# Autodesk Inventor assembly: Carriage
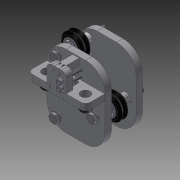
[picture p0: Inventor's stored thumbnail of the model, 180x180]
Saved by Autodesk Inventor 2014 (Build 180170000, 170)
## iProperties
Created: 2014-08-27
Part Number: Carriage
Document SubType Name: Assembly
Designer: ThatOtherGuy
Author: ThatOtherGuy
## Documents named in this file (17)
- U:\Hobbies\Inventor\KosselCNC1515\Carriage\Carriage.iam
- U:\Hobbies\Inventor\KosselCNC1515\Carriage\Carriage_Frame.ipt
- U:\Hobbies\Inventor\KosselCNC1515\Carriage\Carriage_Spacer-6.35mm.ipt
- Carriage_Spacer-6.35mm.ipt
- U:\Hobbies\Inventor\KosselCNC1515\Carriage\OpenVWheel.iam
- U:\Hobbies\Inventor\Content Center Files\R2014\en-US\DIN 125-1  A\DIN 125 - A 5.3.ipt
- U:\Hobbies\Inventor\Content Center Files\R2014\en-US\DIN 125-1  A\DIN 125 - A 4.3.ipt
- U:\Hobbies\Inventor\Content Center Files\R2014\en-US\ISO 10511\ISO 10511 - M5.ipt
- U:\Hobbies\Inventor\KosselCNC1515\Carriage\Carriage_Frame_Back.ipt
- U:\Hobbies\Inventor\KosselCNC1515\Carriage\Carriage_Joint_Frame.ipt
- U:\Hobbies\Inventor\KosselCNC1515\Joints\Joint_Ball_Bearing_12MM.ipt
- U:\Hobbies\Inventor\Content Center Files\R2014\en-US\JIS B 1180  A\JIS B 1180 - A M5 x 50 - 0.8.ipt
- U:\Hobbies\Inventor\KosselCNC1515\Carriage\Carriage_Joint_Boltblock.ipt
- U:\Hobbies\Inventor\KosselCNC1515\Carriage\Carriage_Joint_Boltblock_Brace.ipt
- U:\Hobbies\Inventor\Content Center Files\R2014\en-US\ANSI B18.3.1M(1)\ANSI B18.3.1M - M3x0.5 x 25(2).ipt
- U:\Hobbies\Inventor\Content Center Files\R2014\en-US\DIN 934\DIN 934 - M3 x 0.5.ipt
- U:\Hobbies\Inventor\KosselCNC1515\Carriage\OpenBuilds_Eccentric_Spacer.ipt
## Components (38 placed, 15 different names)
1. Carriage_Frame_Back:1 — Mate:1, Mate:2, Mate:3, Mate:4, Insert:6, Insert:7, Mate:50, Mate:65
2. Carriage_Frame:2 — Mate:26, Mate:27, Mate:28, Insert:4, Insert:5, Mate:45, Mate:46, Mate:60, Mate:65
3. Carriage_Joint_Frame:1 — Mate:45, Mate:46, Mate:60, Mate:71, Mate:72, Tangent:1, Tangent:2, Mate:75, Mate:76, Mate:77
4. Joint_Ball_Bearing_12MM:1 — Mate:71, Tangent:1
5. Joint_Ball_Bearing_12MM:2 — Mate:72, Tangent:2
6. DIN EN ISO 10511 M5:3
7. Carriage_Joint_Boltblock:1 — Mate:75, Mate:76, Mate:77, Mate:78, Mate:79, Mate:80, Insert:18, Insert:19, Insert:20, Insert:21, Angle:1
8. Carriage_Joint_Boltblock_Brace:1 — Mate:78, Mate:79, Mate:80
9. Broached Socket Head Cap Screw - Metric M3x0.5 x 25:1 — Insert:18
10. Broached Socket Head Cap Screw - Metric M3x0.5 x 25:2 — Insert:19
11. DIN 934 - replaced by DIN EN 24032/28673/28674 M3:1 — Insert:20, Angle:1, Angle:2
12. DIN 934 - replaced by DIN EN 24032/28673/28674 M3:2 — Insert:21, Angle:2
13. JIS B 1180 A - Metric A M5 x 50:1 — Mate:73
14. DIN 125-1 A A 5.3:8
15. DIN 125-1 A A 5.3:9
16. OpenBuilds_Eccentric_Spacer:3 — Mate:1, Mate:2, Mate:8, Insert:1, Mate:49
17. OpenVWheel:1 [sub-assembly] — Mate:8, Mate:9, Mate:14, Mate:15, Mate:25
18. DIN 125-1 A A 5.3:1 — Insert:1, Mate:9
19. DIN 125-1 A A 4.3:1 — Mate:14, Mate:15, Mate:24
20. OpenBuilds_Eccentric_Spacer:4 — Mate:24, Mate:25, Mate:26, Mate:27, Mate:49, Mate:73
21. DIN EN ISO 10511 M5:2 — Insert:9, Mate:6
22. JIS B 1180 A - Metric A M5 x 50:3
23. DIN 125-1 A A 5.3:5 — Insert:5
24. DIN 125-1 A A 5.3:7 — Insert:7, Insert:9
25. Carriage_Spacer-6.35mm:1 — Mate:4, Mate:6, Insert:3, Mate:13
26. OpenVWheel:2 [sub-assembly] — Mate:12, Mate:13, Mate:18, Mate:19, Mate:23
27. DIN 125-1 A A 5.3:3 — Insert:3, Mate:12
28. DIN 125-1 A A 4.3:3 — Mate:18, Mate:19, Mate:20
29. Carriage_Spacer-6.35mm:3 — Mate:20, Mate:23
30. DIN EN ISO 10511 M5:1 — Insert:8, Mate:5
31. JIS B 1180 A - Metric A M5 x 50:2 — Mate:36, Mate:50
32. DIN 125-1 A A 5.3:4 — Insert:4, Mate:36
33. DIN 125-1 A A 5.3:6 — Insert:6, Insert:8
34. Carriage_Spacer-6.35mm:2 — Mate:3, Mate:5, Insert:2, Mate:11
35. OpenVWheel:3 [sub-assembly] — Mate:10, Mate:11, Mate:16, Mate:17, Mate:22
36. DIN 125-1 A A 5.3:2 — Insert:2, Mate:10
37. DIN 125-1 A A 4.3:2 — Mate:16, Mate:17, Mate:21
38. Carriage_Spacer-6.35mm:4 — Mate:21, Mate:22, Mate:28
## Relationships (68: Mate 50, Insert 14, Tangent 2, Angle 2)
- Mate:1: Carriage_Frame_Back:1 ↔ OpenBuilds_Eccentric_Spacer:3
- Mate:2: Carriage_Frame_Back:1 ↔ OpenBuilds_Eccentric_Spacer:3
- Mate:3: Carriage_Frame_Back:1 ↔ Carriage_Spacer-6.35mm:2
- Mate:4: Carriage_Frame_Back:1 ↔ Carriage_Spacer-6.35mm:1
- Mate:5: DIN EN ISO 10511 M5:1 ↔ Carriage_Spacer-6.35mm:2
- Mate:6: DIN EN ISO 10511 M5:2 ↔ Carriage_Spacer-6.35mm:1
- Mate:8: OpenBuilds_Eccentric_Spacer:3 ↔ OpenVWheel:1
- Insert:1: OpenBuilds_Eccentric_Spacer:3 ↔ DIN 125-1 A A 5.3:1
- Insert:2: Carriage_Spacer-6.35mm:2 ↔ DIN 125-1 A A 5.3:2
- Insert:3: Carriage_Spacer-6.35mm:1 ↔ DIN 125-1 A A 5.3:3
- Mate:9: OpenVWheel:1 ↔ DIN 125-1 A A 5.3:1
- Mate:10: OpenVWheel:3 ↔ DIN 125-1 A A 5.3:2
- Mate:11: Carriage_Spacer-6.35mm:2 ↔ OpenVWheel:3
- Mate:12: OpenVWheel:2 ↔ DIN 125-1 A A 5.3:3
- Mate:13: Carriage_Spacer-6.35mm:1 ↔ OpenVWheel:2
- Mate:14: OpenVWheel:1 ↔ DIN 125-1 A A 4.3:1
- Mate:15: OpenVWheel:1 ↔ DIN 125-1 A A 4.3:1
- Mate:16: OpenVWheel:3 ↔ DIN 125-1 A A 4.3:2
- Mate:17: OpenVWheel:3 ↔ DIN 125-1 A A 4.3:2
- Mate:18: OpenVWheel:2 ↔ DIN 125-1 A A 4.3:3
- Mate:19: OpenVWheel:2 ↔ DIN 125-1 A A 4.3:3
- Mate:20: DIN 125-1 A A 4.3:3 ↔ Carriage_Spacer-6.35mm:3
- Mate:21: DIN 125-1 A A 4.3:2 ↔ Carriage_Spacer-6.35mm:4
- Mate:22: OpenVWheel:3 ↔ Carriage_Spacer-6.35mm:4
- Mate:23: OpenVWheel:2 ↔ Carriage_Spacer-6.35mm:3
- Mate:24: DIN 125-1 A A 4.3:1 ↔ OpenBuilds_Eccentric_Spacer:4
- Mate:25: OpenVWheel:1 ↔ OpenBuilds_Eccentric_Spacer:4
- Mate:26: Carriage_Frame:2 ↔ OpenBuilds_Eccentric_Spacer:4
- Mate:27: Carriage_Frame:2 ↔ OpenBuilds_Eccentric_Spacer:4
- Mate:28: Carriage_Frame:2 ↔ Carriage_Spacer-6.35mm:4
- Insert:4: Carriage_Frame:2 ↔ DIN 125-1 A A 5.3:4
- Insert:5: Carriage_Frame:2 ↔ DIN 125-1 A A 5.3:5
- Insert:6: Carriage_Frame_Back:1 ↔ DIN 125-1 A A 5.3:6
- Insert:7: Carriage_Frame_Back:1 ↔ DIN 125-1 A A 5.3:7
- [Mate]: Carriage_Frame:2 ↔ JIS B 1180 A - Metric A M5 x 50:2
- Mate:36: JIS B 1180 A - Metric A M5 x 50:2 ↔ DIN 125-1 A A 5.3:4
- [Mate]: Carriage_Frame:2 ↔ JIS B 1180 A - Metric A M5 x 50:3
- Insert:8: DIN EN ISO 10511 M5:1 ↔ DIN 125-1 A A 5.3:6
- Insert:9: DIN EN ISO 10511 M5:2 ↔ DIN 125-1 A A 5.3:7
- Mate:45: Carriage_Frame:2 ↔ Carriage_Joint_Frame:1
- Mate:46: Carriage_Frame:2 ↔ Carriage_Joint_Frame:1
- Mate:49: OpenBuilds_Eccentric_Spacer:3 ↔ OpenBuilds_Eccentric_Spacer:4
- Mate:50: Carriage_Frame_Back:1 ↔ JIS B 1180 A - Metric A M5 x 50:2
- [Mate]: DIN 125-1 A A 5.3:8 ↔ OpenBuilds_Eccentric_Spacer:4
- [Mate]: Carriage_Frame:2 ↔ DIN 125-1 A A 5.3:8
- [Mate]: DIN 125-1 A A 5.3:9 ↔ OpenBuilds_Eccentric_Spacer:3
- [Mate]: Carriage_Frame_Back:1 ↔ DIN 125-1 A A 5.3:9
- Mate:60: Carriage_Frame:2 ↔ Carriage_Joint_Frame:1
- Mate:65: Carriage_Frame_Back:1 ↔ Carriage_Frame:2
- Mate:71: Carriage_Joint_Frame:1 ↔ Joint_Ball_Bearing_12MM:1
- Mate:72: Carriage_Joint_Frame:1 ↔ Joint_Ball_Bearing_12MM:2
- Tangent:1 (-2.35 mm): Carriage_Joint_Frame:1 ↔ Joint_Ball_Bearing_12MM:1
- Tangent:2 (-2.35 mm): Carriage_Joint_Frame:1 ↔ Joint_Ball_Bearing_12MM:2
- Mate:73: JIS B 1180 A - Metric A M5 x 50:1 ↔ OpenBuilds_Eccentric_Spacer:4
- [Mate]: JIS B 1180 A - Metric A M5 x 50:1 ↔ DIN 125-1 A A 5.3:8
- [Insert]: DIN EN ISO 10511 M5:3 ↔ DIN 125-1 A A 5.3:9
- Mate:75: Carriage_Joint_Frame:1 ↔ Carriage_Joint_Boltblock:1
- Mate:76: Carriage_Joint_Frame:1 ↔ Carriage_Joint_Boltblock:1
- Mate:77: Carriage_Joint_Frame:1 ↔ Carriage_Joint_Boltblock:1
- Mate:78: Carriage_Joint_Boltblock:1 ↔ Carriage_Joint_Boltblock_Brace:1
- Mate:79: Carriage_Joint_Boltblock:1 ↔ Carriage_Joint_Boltblock_Brace:1
- Mate:80: Carriage_Joint_Boltblock:1 ↔ Carriage_Joint_Boltblock_Brace:1
- Insert:18: Carriage_Joint_Boltblock:1 ↔ Broached Socket Head Cap Screw - Metric M3x0.5 x 25:1
- Insert:19: Carriage_Joint_Boltblock:1 ↔ Broached Socket Head Cap Screw - Metric M3x0.5 x 25:2
- Insert:20: Carriage_Joint_Boltblock:1 ↔ DIN 934 - replaced by DIN EN 24032/28673/28674 M3:1
- Insert:21: Carriage_Joint_Boltblock:1 ↔ DIN 934 - replaced by DIN EN 24032/28673/28674 M3:2
- Angle:1 (0 deg): Carriage_Joint_Boltblock:1 ↔ DIN 934 - replaced by DIN EN 24032/28673/28674 M3:1
- Angle:2 (0 deg): DIN 934 - replaced by DIN EN 24032/28673/28674 M3:1 ↔ DIN 934 - replaced by DIN EN 24032/28673/28674 M3:2
